# Autodesk Inventor assembly: 000.100 - Часть ходовая
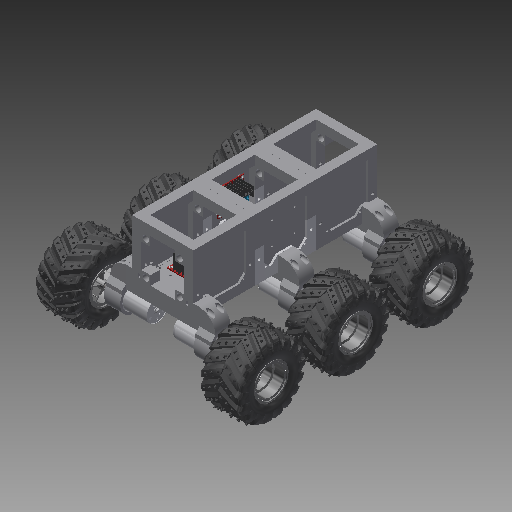
[picture p0: Inventor's stored thumbnail of the model, 512x512]
Saved by Autodesk Inventor 2019 (Build 230136000, 136)
## iProperties
Created: 2020-06-05
Part Number: 000.100 - Часть ходовая
Material: Типовые
Document SubType Name: Assembly
Designer: Петров Иван
Author: Петров Иван
## Documents named in this file (20)
- E:\IVAN\Ivan_desktop\My_projects\RTK\000.100 - Часть ходовая.iam
- E:\IVAN\Ivan_desktop\My_projects\RTK\000.101 - Центральный сегмент ходовой части.ipt
- E:\IVAN\Ivan_desktop\My_projects\RTK\000.102 - Передний сегмент ходовой части - копия.ipt
- E:\IVAN\Ivan_desktop\My_projects\RTK\000.103 - Задний сегмент ходовой части.ipt
- E:\IVAN\Ivan_desktop\My_projects\RTK\000.200 - Средняя ось.iam
- E:\IVAN\Ivan_desktop\My_projects\RTK\000.300 - Передняя ось.iam
- E:\IVAN\Ivan_desktop\My_projects\RTK\000.400 - Задняя ось.iam
- E:\IVAN\Ivan_desktop\My_projects\RTK\000.104 - Дно цетрального сегмента.ipt
- E:\IVAN\Ivan_desktop\My_projects\RTK\000.105 - Дно переднего сегмента.ipt
- E:\IVAN\Ivan_desktop\My_projects\RTK\000.106 - Дно заднего сегмента.ipt
- E:\IVAN\Ivan_desktop\My_projects\RTK\components\L298N_V2.ipt
- E:\IVAN\Ivan_desktop\My_projects\RTK\000.107 - Правая стенка среднего сегмента.ipt
- E:\IVAN\Ivan_desktop\My_projects\RTK\000.108 - Левая стенка среднего сегмента.ipt
- E:\IVAN\Ivan_desktop\My_projects\RTK\000.109 - Правая боковая панель заднего сегмента.ipt
- E:\IVAN\Ivan_desktop\My_projects\RTK\000.110 - Левая боковая панель заднего сегмента.ipt
- E:\IVAN\Ivan_desktop\My_projects\RTK\000.111 - Правая боковая панель переднего сегмента.ipt
- E:\IVAN\Ivan_desktop\My_projects\RTK\000.112 - Левая боковая панель переднего сегмента.ipt
- E:\IVAN\Ivan_desktop\My_projects\RTK\000.113 - Верх центрального сегмента.ipt
- E:\IVAN\Ivan_desktop\My_projects\RTK\000.114 - Верх заднего сегмента.ipt
- E:\IVAN\Ivan_desktop\My_projects\RTK\000.115 - Верх переднего сегмента.ipt
## Components (23 placed, 19 different names)
1. 000.101 - Центральный сегмент ходовой части:1 — Совмещение:1, Совмещение:2, Совмещение:3, Совмещение:4, Совмещение:5, Совмещение:6, Совмещение:8, Совмещение:9, Совмещение:10, Совмещение:17, Совмещение:18, Совмещение:19, Совмещение:39, Совмещение:40, Совмещение:41, Совмещение:45, Совмещение:46, Совмещение:47, Совмещение:63, Заподлицо:1, Заподлицо:2
2. 000.102 - Передний сегмент ходовой части - копия:1 — Совмещение:1, Совмещение:2, Совмещение:3, Совмещение:11, Совмещение:12, Совмещение:13, Совмещение:20, Совмещение:21, Совмещение:22, Совмещение:57, Совмещение:58, Совмещение:59, Совмещение:60, Совмещение:61, Совмещение:62, Совмещение:65, Заподлицо:5, Заподлицо:6
3. 000.103 - Задний сегмент ходовой части:1 — Совмещение:4, Совмещение:5, Совмещение:6, Совмещение:14, Совмещение:15, Совмещение:16, Совмещение:23, Совмещение:24, Совмещение:25, Совмещение:51, Совмещение:52, Совмещение:53, Совмещение:54, Совмещение:55, Совмещение:56, Совмещение:64, Заподлицо:3, Заподлицо:4
4. 000.200 - Средняя ось:1 [sub-assembly] — Совмещение:8, Совмещение:9, Совмещение:10
5. 000.300 - Передняя ось:1 [sub-assembly] — Совмещение:11, Совмещение:12, Совмещение:13
6. 000.400 - Задняя ось:1 [sub-assembly] — Совмещение:14, Совмещение:15, Совмещение:16
7. 000.104 - Дно цетрального сегмента:1 — Совмещение:17, Совмещение:18, Совмещение:19, Совмещение:26, Совмещение:27, Совмещение:28
8. 000.105 - Дно переднего сегмента:1 — Совмещение:20, Совмещение:21, Совмещение:22, Совмещение:29, Совмещение:30, Совмещение:31
9. 000.106 - Дно заднего сегмента:1 — Совмещение:23, Совмещение:24, Совмещение:25, Совмещение:32, Совмещение:33, Совмещение:34
10. L298N_V2:1 — Совмещение:26, Совмещение:27, Совмещение:28
11. L298N_V2:2 — Совмещение:29, Совмещение:30, Совмещение:31
12. L298N_V2:3 — Совмещение:32, Совмещение:33, Совмещение:34
13. L298N_V2:4 — Совмещение:48, Совмещение:49, Совмещение:50
14. L298N_V2:5 — Совмещение:42, Совмещение:43, Совмещение:44
15. 000.107 - Правая стенка среднего сегмента:2 — Совмещение:39, Совмещение:40, Совмещение:41, Совмещение:42, Совмещение:43, Совмещение:44
16. 000.108 - Левая стенка среднего сегмента:1 — Совмещение:45, Совмещение:46, Совмещение:47, Совмещение:48, Совмещение:49, Совмещение:50
17. 000.109 - Правая боковая панель заднего сегмента:1 — Совмещение:51, Совмещение:52, Совмещение:53
18. 000.110 - Левая боковая панель заднего сегмента:1 — Совмещение:54, Совмещение:55, Совмещение:56
19. 000.111 - Правая боковая панель переднего сегмента:1 — Совмещение:57, Совмещение:58, Совмещение:59
20. 000.112 - Левая боковая панель переднего сегмента:1 — Совмещение:60, Совмещение:61, Совмещение:62
21. 000.113 - Верх центрального сегмента:1 — Совмещение:63, Заподлицо:1, Заподлицо:2
22. 000.114 - Верх заднего сегмента:1 — Совмещение:64, Заподлицо:3, Заподлицо:4
23. 000.115 - Верх переднего сегмента:1 — Совмещение:65, Заподлицо:5, Заподлицо:6
## Relationships (66: Mate 60, Flush 6)
- Совмещение:1 [Mate]: 000.101 - Центральный сегмент ходовой части:1 ↔ 000.102 - Передний сегмент ходовой части - копия:1
- Совмещение:2 [Mate]: 000.101 - Центральный сегмент ходовой части:1 ↔ 000.102 - Передний сегмент ходовой части - копия:1
- Совмещение:3 [Mate]: 000.101 - Центральный сегмент ходовой части:1 ↔ 000.102 - Передний сегмент ходовой части - копия:1
- Совмещение:4 [Mate]: 000.101 - Центральный сегмент ходовой части:1 ↔ 000.103 - Задний сегмент ходовой части:1
- Совмещение:5 [Mate]: 000.101 - Центральный сегмент ходовой части:1 ↔ 000.103 - Задний сегмент ходовой части:1
- Совмещение:6 [Mate]: 000.101 - Центральный сегмент ходовой части:1 ↔ 000.103 - Задний сегмент ходовой части:1
- Совмещение:8 [Mate]: 000.101 - Центральный сегмент ходовой части:1 ↔ 000.200 - Средняя ось:1
- Совмещение:9 [Mate]: 000.101 - Центральный сегмент ходовой части:1 ↔ 000.200 - Средняя ось:1
- Совмещение:10 [Mate]: 000.101 - Центральный сегмент ходовой части:1 ↔ 000.200 - Средняя ось:1
- Совмещение:11 [Mate]: 000.102 - Передний сегмент ходовой части - копия:1 ↔ 000.300 - Передняя ось:1
- Совмещение:12 [Mate]: 000.102 - Передний сегмент ходовой части - копия:1 ↔ 000.300 - Передняя ось:1
- Совмещение:13 [Mate]: 000.102 - Передний сегмент ходовой части - копия:1 ↔ 000.300 - Передняя ось:1
- Совмещение:14 [Mate]: 000.103 - Задний сегмент ходовой части:1 ↔ 000.400 - Задняя ось:1
- Совмещение:15 [Mate]: 000.103 - Задний сегмент ходовой части:1 ↔ 000.400 - Задняя ось:1
- Совмещение:16 [Mate]: 000.103 - Задний сегмент ходовой части:1 ↔ 000.400 - Задняя ось:1
- Совмещение:17 [Mate]: 000.101 - Центральный сегмент ходовой части:1 ↔ 000.104 - Дно цетрального сегмента:1
- Совмещение:18 [Mate]: 000.101 - Центральный сегмент ходовой части:1 ↔ 000.104 - Дно цетрального сегмента:1
- Совмещение:19 [Mate]: 000.101 - Центральный сегмент ходовой части:1 ↔ 000.104 - Дно цетрального сегмента:1
- Совмещение:20 [Mate]: 000.102 - Передний сегмент ходовой части - копия:1 ↔ 000.105 - Дно переднего сегмента:1
- Совмещение:21 [Mate]: 000.102 - Передний сегмент ходовой части - копия:1 ↔ 000.105 - Дно переднего сегмента:1
- Совмещение:22 [Mate]: 000.102 - Передний сегмент ходовой части - копия:1 ↔ 000.105 - Дно переднего сегмента:1
- Совмещение:23 [Mate]: 000.103 - Задний сегмент ходовой части:1 ↔ 000.106 - Дно заднего сегмента:1
- Совмещение:24 [Mate]: 000.103 - Задний сегмент ходовой части:1 ↔ 000.106 - Дно заднего сегмента:1
- Совмещение:25 [Mate]: 000.103 - Задний сегмент ходовой части:1 ↔ 000.106 - Дно заднего сегмента:1
- Совмещение:26 [Mate] (10 mm): 000.104 - Дно цетрального сегмента:1 ↔ L298N_V2:1
- Совмещение:27 [Mate]: 000.104 - Дно цетрального сегмента:1 ↔ L298N_V2:1
- Совмещение:28 [Mate]: 000.104 - Дно цетрального сегмента:1 ↔ L298N_V2:1
- Совмещение:29 [Mate] (10 mm): 000.105 - Дно переднего сегмента:1 ↔ L298N_V2:2
- Совмещение:30 [Mate]: 000.105 - Дно переднего сегмента:1 ↔ L298N_V2:2
- Совмещение:31 [Mate]: 000.105 - Дно переднего сегмента:1 ↔ L298N_V2:2
- Совмещение:32 [Mate] (10 mm): 000.106 - Дно заднего сегмента:1 ↔ L298N_V2:3
- Совмещение:33 [Mate]: 000.106 - Дно заднего сегмента:1 ↔ L298N_V2:3
- Совмещение:34 [Mate]: 000.106 - Дно заднего сегмента:1 ↔ L298N_V2:3
- Совмещение:39 [Mate]: 000.101 - Центральный сегмент ходовой части:1 ↔ 000.107 - Правая стенка среднего сегмента:2
- Совмещение:40 [Mate]: 000.101 - Центральный сегмент ходовой части:1 ↔ 000.107 - Правая стенка среднего сегмента:2
- Совмещение:41 [Mate]: 000.101 - Центральный сегмент ходовой части:1 ↔ 000.107 - Правая стенка среднего сегмента:2
- Совмещение:42 [Mate] (4 mm): L298N_V2:5 ↔ 000.107 - Правая стенка среднего сегмента:2
- Совмещение:43 [Mate]: L298N_V2:5 ↔ 000.107 - Правая стенка среднего сегмента:2
- Совмещение:44 [Mate]: L298N_V2:5 ↔ 000.107 - Правая стенка среднего сегмента:2
- Совмещение:45 [Mate]: 000.101 - Центральный сегмент ходовой части:1 ↔ 000.108 - Левая стенка среднего сегмента:1
- Совмещение:46 [Mate]: 000.101 - Центральный сегмент ходовой части:1 ↔ 000.108 - Левая стенка среднего сегмента:1
- Совмещение:47 [Mate]: 000.101 - Центральный сегмент ходовой части:1 ↔ 000.108 - Левая стенка среднего сегмента:1
- Совмещение:48 [Mate] (4 mm): L298N_V2:4 ↔ 000.108 - Левая стенка среднего сегмента:1
- Совмещение:49 [Mate]: L298N_V2:4 ↔ 000.108 - Левая стенка среднего сегмента:1
- Совмещение:50 [Mate]: L298N_V2:4 ↔ 000.108 - Левая стенка среднего сегмента:1
- Совмещение:51 [Mate]: 000.103 - Задний сегмент ходовой части:1 ↔ 000.109 - Правая боковая панель заднего сегмента:1
- Совмещение:52 [Mate]: 000.103 - Задний сегмент ходовой части:1 ↔ 000.109 - Правая боковая панель заднего сегмента:1
- Совмещение:53 [Mate]: 000.103 - Задний сегмент ходовой части:1 ↔ 000.109 - Правая боковая панель заднего сегмента:1
- Совмещение:54 [Mate]: 000.103 - Задний сегмент ходовой части:1 ↔ 000.110 - Левая боковая панель заднего сегмента:1
- Совмещение:55 [Mate]: 000.103 - Задний сегмент ходовой части:1 ↔ 000.110 - Левая боковая панель заднего сегмента:1
- Совмещение:56 [Mate]: 000.103 - Задний сегмент ходовой части:1 ↔ 000.110 - Левая боковая панель заднего сегмента:1
- Совмещение:57 [Mate]: 000.102 - Передний сегмент ходовой части - копия:1 ↔ 000.111 - Правая боковая панель переднего сегмента:1
- Совмещение:58 [Mate]: 000.102 - Передний сегмент ходовой части - копия:1 ↔ 000.111 - Правая боковая панель переднего сегмента:1
- Совмещение:59 [Mate]: 000.102 - Передний сегмент ходовой части - копия:1 ↔ 000.111 - Правая боковая панель переднего сегмента:1
- Совмещение:60 [Mate]: 000.102 - Передний сегмент ходовой части - копия:1 ↔ 000.112 - Левая боковая панель переднего сегмента:1
- Совмещение:61 [Mate]: 000.102 - Передний сегмент ходовой части - копия:1 ↔ 000.112 - Левая боковая панель переднего сегмента:1
- Совмещение:62 [Mate]: 000.102 - Передний сегмент ходовой части - копия:1 ↔ 000.112 - Левая боковая панель переднего сегмента:1
- Совмещение:63 [Mate]: 000.101 - Центральный сегмент ходовой части:1 ↔ 000.113 - Верх центрального сегмента:1
- Заподлицо:1 [Flush]: 000.101 - Центральный сегмент ходовой части:1 ↔ 000.113 - Верх центрального сегмента:1
- Заподлицо:2 [Flush]: 000.101 - Центральный сегмент ходовой части:1 ↔ 000.113 - Верх центрального сегмента:1
- Совмещение:64 [Mate]: 000.103 - Задний сегмент ходовой части:1 ↔ 000.114 - Верх заднего сегмента:1
- Заподлицо:3 [Flush]: 000.103 - Задний сегмент ходовой части:1 ↔ 000.114 - Верх заднего сегмента:1
- Заподлицо:4 [Flush]: 000.103 - Задний сегмент ходовой части:1 ↔ 000.114 - Верх заднего сегмента:1
- Совмещение:65 [Mate]: 000.102 - Передний сегмент ходовой части - копия:1 ↔ 000.115 - Верх переднего сегмента:1
- Заподлицо:5 [Flush]: 000.102 - Передний сегмент ходовой части - копия:1 ↔ 000.115 - Верх переднего сегмента:1
- Заподлицо:6 [Flush]: 000.102 - Передний сегмент ходовой части - копия:1 ↔ 000.115 - Верх переднего сегмента:1
